# Autodesk Inventor assembly: ASM_Micron_ASAP_Indep_bottom
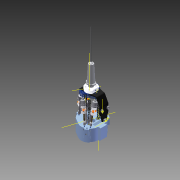
[picture p0: Inventor's stored thumbnail of the model, 180x180]
Saved by Autodesk Inventor 2011 SP2 (Build 150309200, 309)
## iProperties
Created: 2011-08-12
Part Number: ASM_Micron_ASAP_Indep_bottom
Document SubType Name: Assembly
Designer: sungwook
Author: sungwook
## Documents named in this file (10)
- C:\Users\sungwook\Documents\Inventor\Micron22_top_adj_02082013\Assembly\Motion_Merge\Indep\ASM_Micron_ASAP_Indep_bottom.iam
- C:\Users\sungwook\Documents\Inventor\Micron22_top_adj_02082013\Parts\Main\Platform_Base_20mm_Rev2.ipt
- C:\Users\sungwook\Documents\Inventor\Micron22_top_adj_02082013\Parts\Main\Platform_Top_14mm_Rev.ipt
- C:\Users\sungwook\Documents\Inventor\Micron22_top_adj_02082013\Parts\Tool\ASM_Tool_Tip_Rev.iam
- C:\Users\sungwook\Documents\Inventor\Micron22_top_adj_02082013\Parts\ASAP\Platform_ASAP.iam
- C:\Users\sungwook\Documents\Inventor\Micron22_top_adj_02082013\Parts\Main\Spring.ipt
- C:\Users\sungwook\Documents\Inventor\Micron22_top_adj_02082013\Parts\Main\Eye_Pin_26Ga.ipt
- C:\Users\sungwook\Documents\Inventor\Micron22_top_adj_02082013\Assembly\ASM_Motor_Unit_Part1_Rev.iam
- C:\Users\sungwook\Documents\Inventor\Micron22_top_adj_02082013\Assembly\ASM_Motor_Unit_Part2_Rev.iam
- C:\Users\sungwook\Documents\Inventor\Micron22_top_adj_02082013\Param_dMotor.xlsx
## Components (25 placed, 8 different names)
1. Platform_Base_20mm_Rev2:1 — Mate_Top_Bottom, Top_Bottom_Default, Mate:96, Mate:97, Mate:116, Mate:130, Mate:132, Mate:133, Mate:135, Mate:137, Mate:139, Mate:141
2. Platform_Top_14mm_Rev:1 — Mate_Top_Bottom, Mate:20, Mate:21, Mate:22, Top_Bottom_Default, Mate:72, Mate:73, Mate:74, Mate:95, Flush:3, Angle:8, Mate:106, Flush:4, Angle:10, Mate:107, Flush:5, Angle:11, Mate:116, Mate:129, Mate:131, Mate:133, Mate:134, Mate:136, Mate:138, Mate:140
3. ASM_Tool_Tip_Rev:1 [sub-assembly] — Mate:20, Mate:21, Mate:22, Mate:73, Mate:70
4. Platform_ASAP:1 [sub-assembly] — Mate:70, Mate:72, Mate:74
5. Spring:1 — Mate:104, Mate:105
6. Spring:2 — Mate:114, Mate:115
7. Spring:3 — Mate:112, Mate:113
8. Eye_Pin_26Ga:4 — Mate:95, Flush:3, Angle:8, Mate:98, Mate:104
9. Eye_Pin_26Ga:11 — Mate:106, Flush:4, Angle:10, Mate:110, Mate:114
10. Eye_Pin_26Ga:12 — Mate:107, Flush:5, Angle:11, Mate:108, Mate:112
11. ASM_Motor_Unit_Part1_Rev:1 [sub-assembly] — Mate:117, Mate:118, Mate:130
12. ASM_Motor_Unit_Part2_Rev:1 [sub-assembly] — Mate:117, Mate:118, Mate:129
13. ASM_Motor_Unit_Part1_Rev:2 [sub-assembly] — Mate:121, Mate:122, Mate:132
14. ASM_Motor_Unit_Part2_Rev:2 [sub-assembly] — Mate:121, Mate:122, Mate:131
15. ASM_Motor_Unit_Part1_Rev:3 [sub-assembly] — Mate:123, Mate:124, Mate:135
16. ASM_Motor_Unit_Part2_Rev:3 [sub-assembly] — Mate:123, Mate:124, Mate:134
17. ASM_Motor_Unit_Part1_Rev:4 [sub-assembly] — Mate:119, Mate:120, Mate:137
18. ASM_Motor_Unit_Part2_Rev:4 [sub-assembly] — Mate:119, Mate:120, Mate:136
19. ASM_Motor_Unit_Part1_Rev:5 [sub-assembly] — Mate:125, Mate:126, Mate:139
20. ASM_Motor_Unit_Part2_Rev:5 [sub-assembly] — Mate:125, Mate:126, Mate:138
21. ASM_Motor_Unit_Part1_Rev:6 [sub-assembly] — Mate:127, Mate:128, Mate:141
22. ASM_Motor_Unit_Part2_Rev:6 [sub-assembly] — Mate:127, Mate:128, Mate:140
23. Eye_Pin_26Ga:6 — Mate:96, Mate:97, Angle:9, Mate:99
24. Eye_Pin_26Ga:9 — Mate:111
25. Eye_Pin_26Ga:10 — Mate:109
## Component patterns: (3 elements, first: Eye_Pin_26Ga:6)
## Relationships (59: Mate 52, Angle 4, Flush 3)
- Mate_Top_Bottom (30 mm): Platform_Base_20mm_Rev2:1 ↔ Platform_Top_14mm_Rev:1
- Mate:20: Platform_Top_14mm_Rev:1 ↔ ASM_Tool_Tip_Rev:1
- Mate:21: Platform_Top_14mm_Rev:1 ↔ ASM_Tool_Tip_Rev:1
- Mate:22: Platform_Top_14mm_Rev:1 ↔ ASM_Tool_Tip_Rev:1
- Top_Bottom_Default [Mate] (26.2836 mm): Platform_Base_20mm_Rev2:1 ↔ Platform_Top_14mm_Rev:1
- Mate:70: ASM_Tool_Tip_Rev:1 ↔ Platform_ASAP:1
- Mate:72: Platform_Top_14mm_Rev:1 ↔ Platform_ASAP:1
- Mate:73: Platform_Top_14mm_Rev:1 ↔ ASM_Tool_Tip_Rev:1
- Mate:74: Platform_Top_14mm_Rev:1 ↔ Platform_ASAP:1
- Mate:95: Platform_Top_14mm_Rev:1 ↔ Eye_Pin_26Ga:4
- Flush:3: Platform_Top_14mm_Rev:1 ↔ Eye_Pin_26Ga:4
- Angle:8 (0 deg): Platform_Top_14mm_Rev:1 ↔ Eye_Pin_26Ga:4
- Mate:96: Platform_Base_20mm_Rev2:1 ↔ Eye_Pin_26Ga:6
- Mate:97: Platform_Base_20mm_Rev2:1 ↔ Eye_Pin_26Ga:6
- Angle:9 (30 deg): Eye_Pin_26Ga:6
- Mate:98: Eye_Pin_26Ga:4
- Mate:99: Eye_Pin_26Ga:6
- Mate:104: Spring:1 ↔ Eye_Pin_26Ga:4
- Mate:105: Spring:1
- Mate:106: Platform_Top_14mm_Rev:1 ↔ Eye_Pin_26Ga:11
- Flush:4: Platform_Top_14mm_Rev:1 ↔ Eye_Pin_26Ga:11
- Angle:10 (0 deg): Platform_Top_14mm_Rev:1 ↔ Eye_Pin_26Ga:11
- Mate:107: Platform_Top_14mm_Rev:1 ↔ Eye_Pin_26Ga:12
- Flush:5: Platform_Top_14mm_Rev:1 ↔ Eye_Pin_26Ga:12
- Angle:11 (0 deg): Platform_Top_14mm_Rev:1 ↔ Eye_Pin_26Ga:12
- Mate:108: Eye_Pin_26Ga:12
- Mate:109: Eye_Pin_26Ga:10
- Mate:110: Eye_Pin_26Ga:11
- Mate:111: Eye_Pin_26Ga:9
- Mate:112: Spring:3 ↔ Eye_Pin_26Ga:12
- Mate:113: Spring:3
- Mate:114: Spring:2 ↔ Eye_Pin_26Ga:11
- Mate:115: Spring:2
- Mate:116: Platform_Base_20mm_Rev2:1 ↔ Platform_Top_14mm_Rev:1
- Mate:117: ASM_Motor_Unit_Part1_Rev:1 ↔ ASM_Motor_Unit_Part2_Rev:1
- Mate:118: ASM_Motor_Unit_Part1_Rev:1 ↔ ASM_Motor_Unit_Part2_Rev:1
- Mate:119: ASM_Motor_Unit_Part1_Rev:4 ↔ ASM_Motor_Unit_Part2_Rev:4
- Mate:120: ASM_Motor_Unit_Part1_Rev:4 ↔ ASM_Motor_Unit_Part2_Rev:4
- Mate:121: ASM_Motor_Unit_Part1_Rev:2 ↔ ASM_Motor_Unit_Part2_Rev:2
- Mate:122: ASM_Motor_Unit_Part1_Rev:2 ↔ ASM_Motor_Unit_Part2_Rev:2
- Mate:123: ASM_Motor_Unit_Part1_Rev:3 ↔ ASM_Motor_Unit_Part2_Rev:3
- Mate:124: ASM_Motor_Unit_Part1_Rev:3 ↔ ASM_Motor_Unit_Part2_Rev:3
- Mate:125: ASM_Motor_Unit_Part1_Rev:5 ↔ ASM_Motor_Unit_Part2_Rev:5
- Mate:126: ASM_Motor_Unit_Part1_Rev:5 ↔ ASM_Motor_Unit_Part2_Rev:5
- Mate:127: ASM_Motor_Unit_Part1_Rev:6 ↔ ASM_Motor_Unit_Part2_Rev:6
- Mate:128: ASM_Motor_Unit_Part1_Rev:6 ↔ ASM_Motor_Unit_Part2_Rev:6
- Mate:129: Platform_Top_14mm_Rev:1 ↔ ASM_Motor_Unit_Part2_Rev:1
- Mate:130: Platform_Base_20mm_Rev2:1 ↔ ASM_Motor_Unit_Part1_Rev:1
- Mate:131: Platform_Top_14mm_Rev:1 ↔ ASM_Motor_Unit_Part2_Rev:2
- Mate:132: Platform_Base_20mm_Rev2:1 ↔ ASM_Motor_Unit_Part1_Rev:2
- Mate:133: Platform_Base_20mm_Rev2:1 ↔ Platform_Top_14mm_Rev:1
- Mate:134: Platform_Top_14mm_Rev:1 ↔ ASM_Motor_Unit_Part2_Rev:3
- Mate:135: Platform_Base_20mm_Rev2:1 ↔ ASM_Motor_Unit_Part1_Rev:3
- Mate:136: Platform_Top_14mm_Rev:1 ↔ ASM_Motor_Unit_Part2_Rev:4
- Mate:137: Platform_Base_20mm_Rev2:1 ↔ ASM_Motor_Unit_Part1_Rev:4
- Mate:138: Platform_Top_14mm_Rev:1 ↔ ASM_Motor_Unit_Part2_Rev:5
- Mate:139: Platform_Base_20mm_Rev2:1 ↔ ASM_Motor_Unit_Part1_Rev:5
- Mate:140: Platform_Top_14mm_Rev:1 ↔ ASM_Motor_Unit_Part2_Rev:6
- Mate:141: Platform_Base_20mm_Rev2:1 ↔ ASM_Motor_Unit_Part1_Rev:6
## Named parameters: dMotor1 = 0.503 mm, dMotor2 = 0.503 mm, dMotor3 = 0.503 mm, dMotor4 = 0.503 mm, dMotor5 = 0.503 mm, dMotor6 = 0.503 mm
